# Autodesk Inventor assembly: totaal_auto_v2
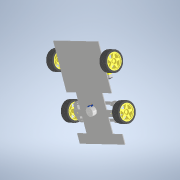
[picture p0: Inventor's stored thumbnail of the model, 180x180]
Saved by Autodesk Inventor 2022 (Build 260153000, 153)
## iProperties
Created: 2021-12-08
Part Number: totaal_auto_v2
Document SubType Name: Assembly
Designer: keemi
Author: keemi
## Documents named in this file (11)
- C:\Users\keemi\OneDrive\Documents\Inventor\Auto\totaal_auto_v2.iam
- C:\Users\keemi\OneDrive\Documents\Inventor\Auto\onderplaat v2.ipt
- C:\Users\keemi\OneDrive\Documents\Inventor\Auto\draaiarm voorwielen.ipt
- C:\Users\keemi\OneDrive\Documents\Inventor\Auto\stuur_arm v2.ipt
- C:\Users\keemi\OneDrive\Documents\Inventor\Auto\wheel-arduino-1.snapshot.2\Wheel ALL.ipt
- C:\Users\keemi\OneDrive\Documents\Inventor\Auto\staafje.ipt
- C:\Users\keemi\OneDrive\Documents\Inventor\Auto\tussenstaaf.ipt
- C:\Users\keemi\OneDrive\Documents\Inventor\Auto\Step - 28BYJ-48.ipt
- C:\Users\keemi\OneDrive\Documents\Inventor\Auto\stuurarm motor.ipt
- C:\Users\keemi\OneDrive\Documents\Inventor\Auto\tussenarmen_sturen.ipt
- C:\Users\keemi\OneDrive\Documents\Inventor\Auto\geared-dc-motor-for-arduino-applications-1.snapshot.2\Hobi - Motor DC 1.ipt
## Components (18 placed, 10 different names)
1. onderplaat v2:1 — Mate:6, Mate:7, Mate:8, Mate:9, Mate:18, Mate:32, Mate:44, Mate:45, Flush:3, Flush:4, Flush:5, Flush:6
2. draaiarm voorwielen:2 — Mate:1, Mate:2, Mate:3, Mate:4, Mate:5
3. stuur_arm v2:1 — Mate:4, Mate:5, Flush:2, Mate:34, Mate:35, Mate:42
4. Wheel ALL:1 — Mate:1, Mate:2, Mate:3
5. staafje:1 — Mate:6, Mate:7, Flush:2, Mate:42
6. staafje:2 — Mate:8, Mate:9, Flush:1, Mate:43
7. draaiarm voorwielen:3
8. stuur_arm v2:2 — Flush:1, Mate:33, Mate:36, Mate:41, Mate:43
9. Wheel ALL:2
10. tussenstaaf:1
11. Step - 28BYJ-48:1 — Mate:18, Mate:32
12. stuurarm motor:1 — Mate:37, Mate:38, Mate:39, Mate:40
13. tussenarmen_sturen:1 — Mate:33, Mate:34, Mate:38, Mate:39, Mate:41
14. tussenarmen_sturen:2 — Mate:35, Mate:36, Mate:37, Mate:40
15. Hobi - Motor DC 1:1 — Mate:45, Flush:3, Flush:6, Mate:47
16. Hobi - Motor DC 1:2 — Mate:44, Flush:4, Flush:5, Mate:46, Mate:48, Mate:49
17. Wheel ALL:3 — Mate:48, Mate:49
18. Wheel ALL:4 — Mate:46, Mate:47
## Relationships (39: Mate 33, Flush 6)
- Mate:1: draaiarm voorwielen:2 ↔ Wheel ALL:1
- Mate:2: draaiarm voorwielen:2 ↔ Wheel ALL:1
- Mate:3: draaiarm voorwielen:2 ↔ Wheel ALL:1
- Mate:4: draaiarm voorwielen:2 ↔ stuur_arm v2:1
- Mate:5: draaiarm voorwielen:2 ↔ stuur_arm v2:1
- Mate:6: onderplaat v2:1 ↔ staafje:1
- Mate:7: onderplaat v2:1 ↔ staafje:1
- Mate:8: onderplaat v2:1 ↔ staafje:2
- Mate:9: onderplaat v2:1 ↔ staafje:2
- [Mate]: draaiarm voorwielen:3 ↔ Wheel ALL:2
- [Mate]: draaiarm voorwielen:3 ↔ Wheel ALL:2
- [Mate]: draaiarm voorwielen:3 ↔ Wheel ALL:2
- [Mate]: draaiarm voorwielen:3 ↔ stuur_arm v2:2
- [Mate]: draaiarm voorwielen:3 ↔ stuur_arm v2:2
- Flush:1: staafje:2 ↔ stuur_arm v2:2
- Flush:2: stuur_arm v2:1 ↔ staafje:1
- Mate:18: onderplaat v2:1 ↔ Step - 28BYJ-48:1
- Mate:32: onderplaat v2:1 ↔ Step - 28BYJ-48:1
- Mate:33: stuur_arm v2:2 ↔ tussenarmen_sturen:1
- Mate:34: stuur_arm v2:1 ↔ tussenarmen_sturen:1
- Mate:35: stuur_arm v2:1 ↔ tussenarmen_sturen:2
- Mate:36: stuur_arm v2:2 ↔ tussenarmen_sturen:2
- Mate:37: stuurarm motor:1 ↔ tussenarmen_sturen:2
- Mate:38: stuurarm motor:1 ↔ tussenarmen_sturen:1
- Mate:39: stuurarm motor:1 ↔ tussenarmen_sturen:1
- Mate:40: stuurarm motor:1 ↔ tussenarmen_sturen:2
- Mate:41: stuur_arm v2:2 ↔ tussenarmen_sturen:1
- Mate:42: stuur_arm v2:1 ↔ staafje:1
- Mate:43: staafje:2 ↔ stuur_arm v2:2
- Mate:44: onderplaat v2:1 ↔ Hobi - Motor DC 1:2
- Mate:45: onderplaat v2:1 ↔ Hobi - Motor DC 1:1
- Flush:3 (50 mm): onderplaat v2:1 ↔ Hobi - Motor DC 1:1
- Flush:4 (50 mm): onderplaat v2:1 ↔ Hobi - Motor DC 1:2
- Flush:5: onderplaat v2:1 ↔ Hobi - Motor DC 1:2
- Flush:6: onderplaat v2:1 ↔ Hobi - Motor DC 1:1
- Mate:46: Hobi - Motor DC 1:2 ↔ Wheel ALL:4
- Mate:47: Hobi - Motor DC 1:1 ↔ Wheel ALL:4
- Mate:48: Hobi - Motor DC 1:2 ↔ Wheel ALL:3
- Mate:49: Hobi - Motor DC 1:2 ↔ Wheel ALL:3
## Named parameters: d12_d6 = 0 mm, d13_d7 = 0 mm, d14_d0 = 0 mm, d15_d1 = 0 mm, d16_d2 = 0 mm
